# Autodesk Inventor assembly: front-tower
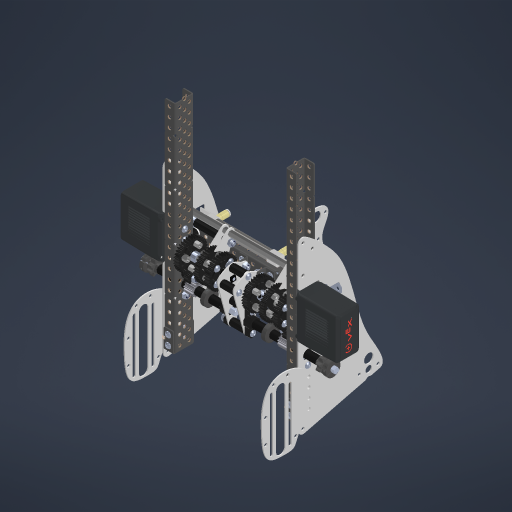
[picture p0: Inventor's stored thumbnail of the model, 512x512]
Saved by Autodesk Inventor 2023 (Build 270158000, 158)
## iProperties
Created: 2023-04-01
Part Number: front-tower
Document SubType Name: Assembly
Designer: Liam
Author: Liam
## Documents named in this file (64)
- C:\Users\eduar\VRC\CAD\Robots\Spin Up\V3\front-tower.iam
- C:\Users\eduar\VRC\CAD\Parts\standard\Structure\C-Channels\1x2x1\C-Channel 1x2x1x23.ipt
- C:\Users\eduar\VRC\CAD\Parts\standard\Structure\U-Channels\U-Channel 2x2x2x1.ipt
- C:\Users\eduar\VRC\CAD\Parts\standard\Structure\Connectors\Nut Thin Nylock.ipt
- C:\Users\eduar\VRC\CAD\Parts\standard\Structure\Connectors\Screw Steel - Star\SScrew Star Smooth .375.ipt
- C:\Users\eduar\VRC\CAD\Parts\custom\plastic\outer-tower-support-proto.ipt
- C:\Users\eduar\VRC\CAD\Parts\custom\plastic\first-stage.ipt
- C:\Users\eduar\VRC\CAD\Parts\standard\Electronics\V5 Motor.ipt
- C:\Users\eduar\VRC\CAD\Parts\standard\Structure\C-Channels\1x2x1\C-Channel 1x2x1x14.ipt
- C:\Users\eduar\VRC\CAD\Parts\standard\Motion\Spacers\Spacer Nylon .375 OD\NSpacer .375 OD x .375.ipt
- C:\Users\eduar\VRC\CAD\Parts\standard\Structure\Connectors\Screw Steel - Star\SScrew Star Smooth .750.ipt
- C:\Users\eduar\VRC\CAD\Parts\standard\Motion\Spacers\Washer Teflon\TWasher .375 OD x .06250.ipt
- C:\Users\eduar\VRC\CAD\Parts\custom\plastic\coffin-v2.ipt
- C:\Users\eduar\VRC\CAD\Parts\standard\Structure\L-Channels\L-Channel 1x1x2.ipt
- C:\Users\eduar\VRC\CAD\Parts\standard\Motion\Adapters\Insert Circle.ipt
- C:\Users\eduar\VRC\CAD\Parts\standard\Motion\Shafts\Shaft LS\Shaft LS 3.0.ipt
- C:\Users\eduar\VRC\CAD\Parts\standard\Motion\Bearings\HS Bearing Flat.ipt
- C:\Users\eduar\VRC\CAD\Parts\standard\Motion\Spacers\Spacer Nylon .375 OD\NSpacer .375 OD x .500.ipt
- C:\Users\eduar\VRC\CAD\Parts\standard\Motion\Spacers\Spacer Nylon .375 OD\NSpacer .375 OD x .250.ipt
- C:\Users\eduar\VRC\CAD\Parts\standard\Motion\Spacers\Washer Teflon\TWasher .375 OD x .04000.ipt
- C:\Users\eduar\VRC\CAD\Parts\standard\Structure\Connectors\Screw Steel - Star\SScrew Star Smooth 1.000.ipt
- C:\Users\eduar\VRC\CAD\Parts\standard\Structure\Connectors\Screw Steel - Star\SScrew Star Smooth 1.500.ipt
- C:\Users\eduar\VRC\CAD\Parts\standard\Motion\Spacers\Spacer Nylon .500 OD\NSpacer White .500 OD x .125.ipt
- C:\Users\eduar\VRC\CAD\Parts\custom\vex\Thin HS 36T Gear, No Insert.ipt
- C:\Users\eduar\VRC\CAD\Parts\standard\Motion\Adapters\Insert Square.ipt
- C:\Users\eduar\VRC\CAD\Parts\standard\Motion\Shafts\Shaft Collar\Shaft Collar Set Screw.iam
- C:\Users\eduar\VRC\CAD\Parts\standard\Motion\Gears\LS\LS 36T Gear.ipt
- C:\Users\eduar\VRC\CAD\Parts\standard\Structure\Standoff\Standoff .25.ipt
- C:\Users\eduar\VRC\CAD\Parts\standard\Motion\Spacers\Washer Teflon\TWasher .375 OD x .03125.ipt
- C:\Users\eduar\VRC\CAD\Parts\standard\Structure\Connectors\Coupler\Coupler Star .5.ipt
- C:\Users\eduar\VRC\CAD\Parts\custom\plastic\gear-interface-v3.ipt
- C:\Users\eduar\VRC\CAD\Parts\standard\Structure\Standoff\Standoff 6.00.ipt
- C:\Users\eduar\VRC\CAD\Parts\standard\Structure\Standoff\Standoff 1.00.ipt
- C:\Users\eduar\VRC\CAD\Parts\standard\Motion\Pneumatics\Reference Parts\Pistons\Double Acting Piston Body.ipt
- C:\Users\eduar\VRC\CAD\Parts\standard\Motion\Pneumatics\Reference Parts\Pistons\Double Acting Piston Rod.ipt
- C:\Users\eduar\VRC\CAD\Parts\standard\Motion\Pneumatics\Cylinder Mount.ipt
- C:\Users\eduar\VRC\CAD\Parts\standard\Motion\Pneumatics\Fitting for Cylinders.ipt
- C:\Users\eduar\VRC\CAD\Parts\standard\Motion\Shafts\Shaft Collar\Shaft Collar No Screw.iam
- C:\Users\eduar\VRC\CAD\Parts\standard\Structure\Connectors\Screw Steel - Star\SScrew Star Smooth 2.250.ipt
- C:\Users\eduar\VRC\CAD\Parts\standard\Structure\Connectors\Screw Steel - Star\SScrew Star Smooth .250.ipt
- C:\Users\eduar\VRC\CAD\Parts\standard\Motion\Spacers\Spacer Nylon .375 OD\NSpacer .375 OD x .125.ipt
- C:\Users\eduar\VRC\CAD\Parts\standard\Structure\Connectors\Screw Steel - Star\SScrew Star Smooth .875.ipt
- C:\Users\eduar\VRC\CAD\Parts\standard\Motion\Gears\LS\LS 12T Gear.ipt
- C:\Users\eduar\VRC\CAD\Parts\standard\Motion\Gears\HS\HS 12T Gear, No Insert.iam
- D:\CAD\Parts\standard\Motion\Gears\HS\HS Gear.iam
- C:\Users\eduar\VRC\CAD\Parts\standard\Motion\Spacers\HS Spacer\HSpacer .0625.ipt
- C:\Users\eduar\VRC\CAD\Parts\standard\Motion\Spacers\HS Spacer\HSpacer .1250.ipt
- C:\Users\eduar\VRC\CAD\Parts\standard\Motion\Shafts\Shaft HS\Shaft HS 5.0 in.ipt
- C:\Users\eduar\VRC\CAD\Parts\standard\Motion\Chain\6P Sprocket\6P 8T Sprocket, No Insert.iam
- C:\Users\eduar\VRC\CAD\Parts\standard\Motion\Spacers\HS Spacer\HSpacer .5000.ipt
- C:\Users\eduar\VRC\CAD\Parts\standard\Motion\Spacers\HS Spacer\HSpacer .2500.ipt
- C:\Users\eduar\VRC\CAD\Parts\standard\Motion\Shafts\Low Profile HS Shaft Collar.ipt
- C:\Users\eduar\VRC\CAD\Parts\custom\plastic\third-stage.ipt
- C:\Users\eduar\VRC\CAD\Parts\standard\Structure\Connectors\Screw Steel - Star.ipt
- C:\Users\eduar\VRC\CAD\Parts\standard\Motion\Spacers\Spacer Nylon .375 OD.ipt
- C:\Users\eduar\VRC\CAD\Parts\standard\Motion\Spacers\Washer Teflon.ipt
- C:\Users\eduar\VRC\CAD\Parts\standard\Motion\Shafts\Shaft LS.ipt
- C:\Users\eduar\VRC\CAD\Parts\standard\Motion\Spacers\Spacer Nylon .500 OD.ipt
- C:\Users\eduar\VRC\CAD\Parts\standard\Motion\Shafts\Shaft Collar.iam
- C:\Users\eduar\VRC\CAD\Parts\standard\Structure\Standoff.ipt
- C:\Users\eduar\VRC\CAD\Parts\standard\Structure\Connectors\Coupler.ipt
- C:\Users\eduar\VRC\CAD\Parts\standard\Motion\Shafts\Shaft HS.ipt
- C:\Users\eduar\VRC\CAD\Parts\standard\Motion\Spacers\HS Spacer.ipt
- C:\Users\eduar\VRC\CAD\Parts\standard\Motion\Chain\6P Sprocket.iam
## Components (262 placed, 51 different names)
1. C-Channel 1x2x1x23:1 — Rigid:1, Rigid:2, Rigid:3, Rigid:4, Rigid:5, Rigid:10, Rigid:12, Rigid:15, Rigid:17, Rigid:18, Rigid:29, Rigid:34, Rigid:35, Rigid:134, Mate:3, Mate:4, Rigid:224, Rigid:226, Rotational:14, Rigid:235
2. U-Channel 2x2x2x1:2 — Rigid:1, Rigid:6, Rigid:7, Rigid:8, Rigid:9
3. Nut Thin Nylock:1 — Rigid:3
4. Nut Thin Nylock:2 — Rigid:2
5. Nut Thin Nylock:3 — Rigid:4
6. Nut Thin Nylock:4 — Rigid:5
7. SScrew Star Smooth .375:1 — Rigid:6
8. SScrew Star Smooth .375:2 — Rigid:8
9. SScrew Star Smooth .375:3 — Rigid:7
10. SScrew Star Smooth .375:4 — Rigid:9
11. outer-tower-support-proto:1 — Rigid:10, Rigid:178, Rigid:179, Angle:3, Rigid:228, Rigid:241, Rigid:266
12. C-Channel 1x2x1x23:2 — Rigid:12, Rigid:13, Rigid:16, Rigid:19, Rigid:20, Rigid:36, Rigid:37, Rigid:42, Rigid:43, Rigid:44, Rigid:45, Rigid:46, Rigid:100, Mate:1, Mate:2, Rigid:215, Rigid:232, Rotational:13, Rigid:236
13. outer-tower-support-proto:2 — Rigid:13, Rotational:7, Rigid:180, Rigid:230, Rigid:242, Rigid:265
14. V5 Motor:1 — Rigid:16
15. V5 Motor:2 — Rigid:15
16. SScrew Star Smooth .375:5 — Rigid:17
17. SScrew Star Smooth .375:6 — Rigid:18
18. SScrew Star Smooth .375:7 — Rigid:19
19. SScrew Star Smooth .375:8 — Rigid:20
20. C-Channel 1x2x1x14:1 — Rigid:29, Rigid:30, Rigid:31, Rigid:32, Rigid:33, Rigid:47, Rigid:48, Rigid:63, Rigid:64, Rigid:65, Rigid:66, Angle:4, Rigid:263
21. Nut Thin Nylock:5
22. Nut Thin Nylock:6
23. Nut Thin Nylock:7
24. Nut Thin Nylock:8
25. NSpacer .375 OD x .375:1
26. SScrew Star Smooth .750:9 — Rigid:34
27. SScrew Star Smooth .750:10 — Rigid:35
28. SScrew Star Smooth .750:11 — Rigid:36
29. SScrew Star Smooth .750:12 — Rigid:37
30. TWasher .375 OD x .06250:1 — Rigid:30
31. NSpacer .375 OD x .375:2
32. TWasher .375 OD x .06250:2 — Rigid:33
33. NSpacer .375 OD x .375:3
34. TWasher .375 OD x .06250:3 — Rigid:32
35. NSpacer .375 OD x .375:4
36. TWasher .375 OD x .06250:4 — Rigid:31
37. U-Channel 2x2x2x1:3 — Rigid:42
38. Nut Thin Nylock:9 — Rigid:44
39. Nut Thin Nylock:10 — Rigid:43
40. Nut Thin Nylock:11 — Rigid:45
41. Nut Thin Nylock:12 — Rigid:46
42. SScrew Star Smooth .375:13
43. SScrew Star Smooth .375:14
44. SScrew Star Smooth .375:15
45. SScrew Star Smooth .375:16
46. coffin-v2:1 — Rigid:50, Rigid:61, Rigid:67, Rigid:69, Rigid:202, Rigid:203, Rigid:204, Rigid:207, Rigid:208, Rigid:209, Rigid:210, Rigid:213, Rigid:214
47. coffin-v2:2 — Rigid:49, Rigid:68, Rigid:70, Rigid:74, Rigid:75, Rigid:76, Rigid:211, Rigid:212
48. L-Channel 1x1x2:1 — Rigid:47, Rigid:50, Rigid:51, Rigid:52, Rigid:53, Rigid:54
49. L-Channel 1x1x2:2 — Rigid:48, Rigid:49, Rigid:55, Rigid:56, Rigid:57, Rigid:58
50. SScrew Star Smooth .375:17 — Rigid:52
51. SScrew Star Smooth .375:18 — Rigid:54
52. SScrew Star Smooth .375:19 — Rigid:51
53. SScrew Star Smooth .375:20 — Rigid:53
54. SScrew Star Smooth .375:21 — Rigid:57
55. SScrew Star Smooth .375:22 — Rigid:58
56. SScrew Star Smooth .375:23 — Rigid:56
57. SScrew Star Smooth .375:24 — Rigid:55
58. Nut Thin Nylock:13 — Rigid:210
59. Nut Thin Nylock:14 — Rigid:61
60. Nut Thin Nylock:15 — Rigid:211
61. Nut Thin Nylock:16 — Rigid:212
62. Nut Thin Nylock:17 — Rigid:64
63. Nut Thin Nylock:18 — Rigid:66
64. Nut Thin Nylock:19 — Rigid:63
65. Nut Thin Nylock:20 — Rigid:65
66. Insert Circle:1 — Rigid:67, Rotational:2, Rigid:151
67. Insert Circle:2 — Rigid:68, Rotational:1, Rigid:122
68. Shaft LS 3.0:1 — Rotational:1, Rigid:102, Angle:1, Rigid:127
69. Shaft LS 3.0:2 — Rotational:2, Rigid:135, Angle:2, Rigid:152
70. HS Bearing Flat:1 — Rigid:69, Rigid:97, Rigid:98, Rotational:17
71. HS Bearing Flat:2 — Rigid:70, Rigid:71, Rigid:72, Rotational:18
72. Nut Thin Nylock:21 — Rigid:71
73. Nut Thin Nylock:22 — Rigid:72
74. Nut Thin Nylock:23 — Rigid:76
75. Nut Thin Nylock:24 — Rigid:75
76. Nut Thin Nylock:26 — Rigid:74
77. NSpacer .375 OD x .500:5
78. NSpacer .375 OD x .250:6
79. TWasher .375 OD x .04000:5 — Rigid:208
80. NSpacer .375 OD x .500:7
81. NSpacer .375 OD x .250:8
82. TWasher .375 OD x .04000:6 — Rigid:213
83. NSpacer .375 OD x .500:9
84. NSpacer .375 OD x .250:10
85. TWasher .375 OD x .04000:7 — Rigid:214
86. NSpacer .375 OD x .500:11
87. NSpacer .375 OD x .250:12
88. TWasher .375 OD x .04000:8 — Rigid:207
89. NSpacer .375 OD x .500:13
90. NSpacer .375 OD x .250:14
91. TWasher .375 OD x .04000:9 — Rigid:209
92. SScrew Star Smooth 1.000:25 — Rigid:202
93. SScrew Star Smooth 1.000:26 — Rigid:203
94. SScrew Star Smooth 1.000:27 — Rigid:204
95. SScrew Star Smooth 1.500:29 — Rigid:97
96. SScrew Star Smooth 1.500:30 — Rigid:98
97. NSpacer White .500 OD x .125:1 — Rigid:100
98. TWasher .375 OD x .06250:10 — Rotational:3
99. Thin HS 36T Gear, No Insert:1 — Rigid:101, Rotational:3, Rigid:103, Rigid:104, Rigid:105, Rigid:106, Rigid:153, Rigid:154, Rigid:155, Rigid:156
100. Insert Square:1 — Rigid:101
101. Shaft Collar Set Screw:1 [sub-assembly] — Rigid:102
102. LS 36T Gear:2 — Angle:1, Mate:1, Rigid:107, Rigid:108, Rigid:109, Rigid:110, Rigid:111, Rigid:112, Rigid:113, Rigid:114, Mate:2, Insert:1, Mate:6, Mate:8, Mate:9
103. Standoff .25:1 — Rigid:105
104. Standoff .25:2 — Rigid:106
105. Standoff .25:3 — Rigid:104
106. Standoff .25:4 — Rigid:112, Rigid:169
107. Standoff .25:5 — Rigid:103
108. Standoff .25:6 — Rigid:107
109. Standoff .25:7 — Rigid:111, Rigid:170
110. Standoff .25:8 — Rigid:113, Rigid:172
111. Standoff .25:9 — Rigid:109
112. Standoff .25:10 — Rigid:110
113. Standoff .25:11 — Rigid:114, Rigid:171
114. Standoff .25:12 — Rigid:108
115. Thin HS 36T Gear, No Insert:2 — Rigid:123, Rigid:124, Rigid:125, Rigid:126, Rigid:157, Rigid:158, Rigid:159, Rigid:160
116. Insert Square:2 — Rotational:4
117. NSpacer .375 OD x .250:15 — Rotational:4
118. TWasher .375 OD x .04000:11
119. TWasher .375 OD x .03125:12 — Rigid:122
120. Standoff .25:13 — Rigid:123
121. Standoff .25:14 — Rigid:126
122. Standoff .25:15 — Rigid:124
123. Standoff .25:16 — Rigid:125
124. Shaft Collar Set Screw:2 [sub-assembly] — Rigid:127
125. NSpacer White .500 OD x .125:2 — Rigid:134
126. TWasher .375 OD x .06250:13
127. Thin HS 36T Gear, No Insert:3 — Rigid:165, Rigid:166, Rigid:167, Rigid:168
128. Insert Square:3
129. Standoff .25:17
130. Standoff .25:18
131. Standoff .25:19
132. Standoff .25:20
133. Shaft Collar Set Screw:3 [sub-assembly] — Rigid:135
134. LS 36T Gear:3 — Mate:3, Angle:2, Mate:4, Mate:10, Mate:12, Mate:13, Mate:15
135. Standoff .25:21 — Rigid:174
136. Standoff .25:22
137. Standoff .25:23
138. Standoff .25:24 — Rigid:173
139. Standoff .25:25
140. Standoff .25:26
141. Standoff .25:27 — Rigid:176
142. Standoff .25:28
143. Thin HS 36T Gear, No Insert:4 — Rigid:161, Rigid:162, Rigid:163, Rigid:164
144. Insert Square:4
145. NSpacer .375 OD x .250:16
146. TWasher .375 OD x .04000:14
147. TWasher .375 OD x .03125:15 — Rigid:151
148. Standoff .25:29
149. Standoff .25:30
150. Standoff .25:31 — Rigid:175
151. Standoff .25:32
152. Shaft Collar Set Screw:4 [sub-assembly] — Rigid:152
153. SScrew Star Smooth .375:31 — Rigid:153
154. SScrew Star Smooth .375:32 — Rigid:154
155. SScrew Star Smooth .375:33 — Rigid:155
156. SScrew Star Smooth .375:34 — Rigid:156
157. SScrew Star Smooth .375:35 — Rigid:159
158. SScrew Star Smooth .375:36 — Rigid:160
159. SScrew Star Smooth .375:37 — Rigid:157
160. SScrew Star Smooth .375:38 — Rigid:158
161. SScrew Star Smooth .375:39 — Rigid:161
162. SScrew Star Smooth .375:40 — Rigid:162
163. SScrew Star Smooth .375:41 — Rigid:164
164. SScrew Star Smooth .375:42 — Rigid:163
165. SScrew Star Smooth .375:43 — Rigid:167
166. SScrew Star Smooth .375:44 — Rigid:166
167. SScrew Star Smooth .375:45 — Rigid:165
168. SScrew Star Smooth .375:46 — Rigid:168
169. Coupler Star .5:1 — Rigid:172
170. Coupler Star .5:2 — Rigid:171
171. Coupler Star .5:3 — Rigid:170
172. Coupler Star .5:4 — Rigid:169
173. Coupler Star .5:5 — Rigid:173
174. Coupler Star .5:6 — Rigid:174
175. Coupler Star .5:7 — Rigid:175
176. Coupler Star .5:8 — Rigid:176
177. gear-interface-v3:1 — Insert:1, Mate:5, Mate:9, Rigid:182, Rigid:183
178. Standoff 6.00:33 — Rotational:7, Mate:5, Mate:7, Mate:11, Mate:14, Rigid:177
179. gear-interface-v3:2 — Mate:6, Mate:7, Mate:8, Mate:20, Mate:22
180. gear-interface-v3:3 — Mate:10, Mate:11, Mate:12, Rigid:184
181. gear-interface-v3:4 — Mate:13, Mate:14, Mate:15, Rigid:181, Mate:21
182. Standoff 1.00:34 — Rigid:177
183. NSpacer White .500 OD x .125:3 — Rigid:178
184. SScrew Star Smooth .375:47 — Rigid:179
185. SScrew Star Smooth .375:48 — Rigid:180
186. NSpacer .375 OD x .250:17 — Rigid:181
187. NSpacer .375 OD x .250:18 — Rigid:182
188. Nut Thin Nylock:28 — Rigid:184
189. Nut Thin Nylock:29 — Rigid:183
190. Double Acting Piston Body:1 — Rigid:185, Rigid:186, Angle:4, Rigid:187, Rigid:199
191. Double Acting Piston Rod:1 — Rotational:8
192. Cylinder Mount:1 — Rotational:8, Angle:3, Mate:18
193. Fitting for Cylinders:1 — Rigid:185
194. Fitting for Cylinders:2 — Rigid:186
195. Shaft Collar No Screw:5 [sub-assembly] — Rigid:187, Mate:19, Mate:20, Mate:22, Rigid:189, Rigid:197
196. Shaft Collar No Screw:6 [sub-assembly] — Mate:18, Mate:19, Mate:21, Rigid:188, Rigid:192, Rigid:198
197. SScrew Star Smooth 2.250:49 — Rigid:188
198. SScrew Star Smooth 2.250:50 — Rigid:189
199. NSpacer .375 OD x .375:19 — Rigid:191, Rigid:193
200. NSpacer .375 OD x .500:20 — Rigid:190, Rigid:192
201. NSpacer .375 OD x .500:21 — Rigid:190, Rigid:191
202. TWasher .375 OD x .04000:16 — Rigid:193
203. NSpacer .375 OD x .375:22
204. NSpacer .375 OD x .500:23 — Rigid:197
205. NSpacer .375 OD x .500:24
206. TWasher .375 OD x .04000:17
207. SScrew Star Smooth .250:51 — Rigid:198
208. SScrew Star Smooth .250:52 — Rigid:199
209. HS Bearing Flat:5 — Rigid:215, Rigid:216, Rigid:219, Rigid:246
210. Nut Thin Nylock:30 — Rigid:216, Rigid:217
211. NSpacer .375 OD x .125:25 — Rigid:217
212. Nut Thin Nylock:31 — Rigid:219
213. NSpacer .375 OD x .125:26
214. HS Bearing Flat:6 — Rigid:224, Rigid:251
215. Nut Thin Nylock:32
216. NSpacer .375 OD x .125:27
217. Nut Thin Nylock:33
218. NSpacer .375 OD x .125:28
219. Nut Thin Nylock:35 — Rigid:226
220. SScrew Star Smooth .875:54 — Rigid:228
221. SScrew Star Smooth .875:56 — Rigid:230
222. Nut Thin Nylock:37 — Rigid:232
223. LS 12T Gear:1 — Rotational:13, Rotational:15
224. LS 12T Gear:2 — Rotational:14, Rotational:16
225. Nut Thin Nylock:38 — Rotational:15
226. Nut Thin Nylock:39 — Rotational:16
227. HS 12T Gear, No Insert:1 [sub-assembly] — Rigid:238, Rigid:244, Rigid:254
228. HS 12T Gear, No Insert:2 [sub-assembly] — Rigid:240, Rigid:243, Rigid:253
229. NSpacer .375 OD x .125:29 — Rigid:235
230. NSpacer .375 OD x .125:30 — Rigid:236
231. HSpacer .0625:1 — Rigid:237
232. HSpacer .1250:2 — Rigid:237, Rigid:238
233. HSpacer .0625:3
234. HSpacer .1250:4 — Rigid:240
235. SScrew Star Smooth 1.500:57 — Rigid:242
236. SScrew Star Smooth 1.500:58 — Rigid:241
237. Shaft HS 5.0 in:2 — Rotational:17, Rigid:244, Rigid:250, Rigid:252
238. Shaft HS 5.0 in:3 — Rotational:18, Rigid:243, Rigid:245, Rigid:248
239. 6P 8T Sprocket, No Insert:1 [sub-assembly] — Rigid:245
240. HSpacer .5000:5 — Rigid:246, Rigid:247
241. HSpacer .2500:6 — Rigid:247, Rotational:19
242. HSpacer .1250:7 — Rotational:19
243. Low Profile HS Shaft Collar:1 — Rigid:248
244. 6P 8T Sprocket, No Insert:2 [sub-assembly] — Rigid:250
245. HSpacer .5000:8 — Rigid:251
246. HSpacer .2500:9
247. HSpacer .1250:10
248. Low Profile HS Shaft Collar:2 — Rigid:252
249. HSpacer .5000:11 — Rigid:253, Rigid:255
250. HSpacer .5000:12 — Rigid:254, Rigid:256
251. Low Profile HS Shaft Collar:3 — Rigid:255, Rigid:257
252. Low Profile HS Shaft Collar:4 — Rigid:256, Rigid:262
253. HSpacer .5000:13 — Rigid:257, Rigid:258
254. HSpacer .1250:14 — Rigid:258, Rigid:259
255. HSpacer .0625:15 — Rigid:259
256. HSpacer .5000:16 — Rigid:262
257. HSpacer .1250:17
258. HSpacer .0625:18
259. L-Channel 1x1x2:3 — Rigid:263, Rigid:264
260. third-stage:1 — Rigid:264
261. first-stage:3 — Rigid:265
262. first-stage:4 — Rigid:266
## Relationships (279: WeldJoint 236, Mate 22, RevoluteJoint 16, Angle 4, Insert 1)
- Rigid:1 [WeldJoint]: C-Channel 1x2x1x23:1 ↔ U-Channel 2x2x2x1:2
- Rigid:2 [WeldJoint]: C-Channel 1x2x1x23:1 ↔ Nut Thin Nylock:2
- Rigid:3 [WeldJoint]: C-Channel 1x2x1x23:1 ↔ Nut Thin Nylock:1
- Rigid:4 [WeldJoint]: C-Channel 1x2x1x23:1 ↔ Nut Thin Nylock:3
- Rigid:5 [WeldJoint]: C-Channel 1x2x1x23:1 ↔ Nut Thin Nylock:4
- Rigid:6 [WeldJoint]: U-Channel 2x2x2x1:2 ↔ SScrew Star Smooth .375:1
- Rigid:7 [WeldJoint]: U-Channel 2x2x2x1:2 ↔ SScrew Star Smooth .375:3
- Rigid:8 [WeldJoint]: U-Channel 2x2x2x1:2 ↔ SScrew Star Smooth .375:2
- Rigid:9 [WeldJoint]: U-Channel 2x2x2x1:2 ↔ SScrew Star Smooth .375:4
- Rigid:10 [WeldJoint] (14.2875 mm): C-Channel 1x2x1x23:1 ↔ outer-tower-support-proto:1
- Rigid:12 [WeldJoint] (149.225 mm): C-Channel 1x2x1x23:1 ↔ C-Channel 1x2x1x23:2
- Rigid:13 [WeldJoint] (14.2875 mm): C-Channel 1x2x1x23:2 ↔ outer-tower-support-proto:2
- Rigid:15 [WeldJoint]: C-Channel 1x2x1x23:1 ↔ V5 Motor:2
- Rigid:16 [WeldJoint]: C-Channel 1x2x1x23:2 ↔ V5 Motor:1
- Rigid:17 [WeldJoint]: C-Channel 1x2x1x23:1 ↔ SScrew Star Smooth .375:5
- Rigid:18 [WeldJoint]: C-Channel 1x2x1x23:1 ↔ SScrew Star Smooth .375:6
- Rigid:19 [WeldJoint]: C-Channel 1x2x1x23:2 ↔ SScrew Star Smooth .375:7
- Rigid:20 [WeldJoint]: C-Channel 1x2x1x23:2 ↔ SScrew Star Smooth .375:8
- [WeldJoint]: C-Channel 1x2x1x14:1 ↔ Nut Thin Nylock:5
- [WeldJoint]: C-Channel 1x2x1x14:1 ↔ Nut Thin Nylock:6
- [WeldJoint]: C-Channel 1x2x1x14:1 ↔ Nut Thin Nylock:7
- [WeldJoint]: C-Channel 1x2x1x14:1 ↔ Nut Thin Nylock:8
- [WeldJoint]: NSpacer .375 OD x .375:1 ↔ TWasher .375 OD x .06250:1
- [WeldJoint]: NSpacer .375 OD x .375:2 ↔ TWasher .375 OD x .06250:2
- [WeldJoint]: NSpacer .375 OD x .375:3 ↔ TWasher .375 OD x .06250:3
- [WeldJoint]: NSpacer .375 OD x .375:4 ↔ TWasher .375 OD x .06250:4
- Rigid:29 [WeldJoint] (11.1125 mm): C-Channel 1x2x1x23:1 ↔ C-Channel 1x2x1x14:1
- Rigid:30 [WeldJoint]: C-Channel 1x2x1x14:1 ↔ TWasher .375 OD x .06250:1
- Rigid:31 [WeldJoint]: C-Channel 1x2x1x14:1 ↔ TWasher .375 OD x .06250:4
- Rigid:32 [WeldJoint]: C-Channel 1x2x1x14:1 ↔ TWasher .375 OD x .06250:3
- Rigid:33 [WeldJoint]: C-Channel 1x2x1x14:1 ↔ TWasher .375 OD x .06250:2
- Rigid:34 [WeldJoint]: C-Channel 1x2x1x23:1 ↔ SScrew Star Smooth .750:9
- Rigid:35 [WeldJoint]: C-Channel 1x2x1x23:1 ↔ SScrew Star Smooth .750:10
- Rigid:36 [WeldJoint]: C-Channel 1x2x1x23:2 ↔ SScrew Star Smooth .750:11
- Rigid:37 [WeldJoint]: C-Channel 1x2x1x23:2 ↔ SScrew Star Smooth .750:12
- [WeldJoint]: U-Channel 2x2x2x1:3 ↔ SScrew Star Smooth .375:13
- [WeldJoint]: U-Channel 2x2x2x1:3 ↔ SScrew Star Smooth .375:15
- [WeldJoint]: U-Channel 2x2x2x1:3 ↔ SScrew Star Smooth .375:14
- [WeldJoint]: U-Channel 2x2x2x1:3 ↔ SScrew Star Smooth .375:16
- Rigid:42 [WeldJoint]: C-Channel 1x2x1x23:2 ↔ U-Channel 2x2x2x1:3
- Rigid:43 [WeldJoint]: C-Channel 1x2x1x23:2 ↔ Nut Thin Nylock:10
- Rigid:44 [WeldJoint]: C-Channel 1x2x1x23:2 ↔ Nut Thin Nylock:9
- Rigid:45 [WeldJoint]: C-Channel 1x2x1x23:2 ↔ Nut Thin Nylock:11
- Rigid:46 [WeldJoint]: C-Channel 1x2x1x23:2 ↔ Nut Thin Nylock:12
- Rigid:47 [WeldJoint]: C-Channel 1x2x1x14:1 ↔ L-Channel 1x1x2:1
- Rigid:48 [WeldJoint]: C-Channel 1x2x1x14:1 ↔ L-Channel 1x1x2:2
- Rigid:49 [WeldJoint]: coffin-v2:2 ↔ L-Channel 1x1x2:2
- Rigid:50 [WeldJoint]: coffin-v2:1 ↔ L-Channel 1x1x2:1
- Rigid:51 [WeldJoint]: L-Channel 1x1x2:1 ↔ SScrew Star Smooth .375:19
- Rigid:52 [WeldJoint]: L-Channel 1x1x2:1 ↔ SScrew Star Smooth .375:17
- Rigid:53 [WeldJoint]: L-Channel 1x1x2:1 ↔ SScrew Star Smooth .375:20
- Rigid:54 [WeldJoint]: L-Channel 1x1x2:1 ↔ SScrew Star Smooth .375:18
- Rigid:55 [WeldJoint]: L-Channel 1x1x2:2 ↔ SScrew Star Smooth .375:24
- Rigid:56 [WeldJoint]: L-Channel 1x1x2:2 ↔ SScrew Star Smooth .375:23
- Rigid:57 [WeldJoint]: L-Channel 1x1x2:2 ↔ SScrew Star Smooth .375:21
- Rigid:58 [WeldJoint]: L-Channel 1x1x2:2 ↔ SScrew Star Smooth .375:22
- Rigid:61 [WeldJoint]: coffin-v2:1 ↔ Nut Thin Nylock:14
- Rigid:63 [WeldJoint]: C-Channel 1x2x1x14:1 ↔ Nut Thin Nylock:19
- Rigid:64 [WeldJoint]: C-Channel 1x2x1x14:1 ↔ Nut Thin Nylock:17
- Rigid:65 [WeldJoint]: C-Channel 1x2x1x14:1 ↔ Nut Thin Nylock:20
- Rigid:66 [WeldJoint]: C-Channel 1x2x1x14:1 ↔ Nut Thin Nylock:18
- Rigid:67 [WeldJoint]: coffin-v2:1 ↔ Insert Circle:1
- Rigid:68 [WeldJoint]: coffin-v2:2 ↔ Insert Circle:2
- Rotational:1 [RevoluteJoint]: Insert Circle:2 ↔ Shaft LS 3.0:1
- Rotational:2 [RevoluteJoint]: Insert Circle:1 ↔ Shaft LS 3.0:2
- Rigid:69 [WeldJoint]: coffin-v2:1 ↔ HS Bearing Flat:1
- Rigid:70 [WeldJoint]: coffin-v2:2 ↔ HS Bearing Flat:2
- Rigid:71 [WeldJoint]: HS Bearing Flat:2 ↔ Nut Thin Nylock:21
- Rigid:72 [WeldJoint]: HS Bearing Flat:2 ↔ Nut Thin Nylock:22
- Rigid:74 [WeldJoint]: coffin-v2:2 ↔ Nut Thin Nylock:26
- Rigid:75 [WeldJoint]: coffin-v2:2 ↔ Nut Thin Nylock:24
- Rigid:76 [WeldJoint]: coffin-v2:2 ↔ Nut Thin Nylock:23
- [WeldJoint]: NSpacer .375 OD x .500:5 ↔ NSpacer .375 OD x .250:6
- [WeldJoint]: NSpacer .375 OD x .250:6 ↔ TWasher .375 OD x .04000:5
- [WeldJoint]: NSpacer .375 OD x .500:7 ↔ NSpacer .375 OD x .250:8
- [WeldJoint]: NSpacer .375 OD x .250:8 ↔ TWasher .375 OD x .04000:6
- [WeldJoint]: NSpacer .375 OD x .500:9 ↔ NSpacer .375 OD x .250:10
- [WeldJoint]: NSpacer .375 OD x .250:10 ↔ TWasher .375 OD x .04000:7
- [WeldJoint]: NSpacer .375 OD x .500:11 ↔ NSpacer .375 OD x .250:12
- [WeldJoint]: NSpacer .375 OD x .250:12 ↔ TWasher .375 OD x .04000:8
- [WeldJoint]: NSpacer .375 OD x .500:13 ↔ NSpacer .375 OD x .250:14
- [WeldJoint]: NSpacer .375 OD x .250:14 ↔ TWasher .375 OD x .04000:9
- Rigid:97 [WeldJoint]: HS Bearing Flat:1 ↔ SScrew Star Smooth 1.500:29
- Rigid:98 [WeldJoint]: HS Bearing Flat:1 ↔ SScrew Star Smooth 1.500:30
- [WeldJoint]: NSpacer White .500 OD x .125:1 ↔ TWasher .375 OD x .06250:10
- Rigid:100 [WeldJoint]: C-Channel 1x2x1x23:2 ↔ NSpacer White .500 OD x .125:1
- Rigid:101 [WeldJoint] (-3.175 mm): Thin HS 36T Gear, No Insert:1 ↔ Insert Square:1
- Rotational:3 [RevoluteJoint] (3.175 mm): TWasher .375 OD x .06250:10 ↔ Thin HS 36T Gear, No Insert:1
- Rigid:102 [WeldJoint] (-54.5084 mm): Shaft LS 3.0:1 ↔ Shaft Collar Set Screw:1
- Angle:1 (0 deg): Shaft LS 3.0:1 ↔ LS 36T Gear:2
- Mate:1: C-Channel 1x2x1x23:2 ↔ LS 36T Gear:2
- Rigid:103 [WeldJoint]: Thin HS 36T Gear, No Insert:1 ↔ Standoff .25:5
- Rigid:104 [WeldJoint]: Thin HS 36T Gear, No Insert:1 ↔ Standoff .25:3
- Rigid:105 [WeldJoint]: Thin HS 36T Gear, No Insert:1 ↔ Standoff .25:1
- Rigid:106 [WeldJoint]: Thin HS 36T Gear, No Insert:1 ↔ Standoff .25:2
- Rigid:107 [WeldJoint]: LS 36T Gear:2 ↔ Standoff .25:6
- Rigid:108 [WeldJoint]: LS 36T Gear:2 ↔ Standoff .25:12
- Rigid:109 [WeldJoint]: LS 36T Gear:2 ↔ Standoff .25:9
- Rigid:110 [WeldJoint]: LS 36T Gear:2 ↔ Standoff .25:10
- Rigid:111 [WeldJoint]: LS 36T Gear:2 ↔ Standoff .25:7
- Rigid:112 [WeldJoint]: LS 36T Gear:2 ↔ Standoff .25:4
- Rigid:113 [WeldJoint]: LS 36T Gear:2 ↔ Standoff .25:8
- Rigid:114 [WeldJoint]: LS 36T Gear:2 ↔ Standoff .25:11
- [WeldJoint] (-3.175 mm): Thin HS 36T Gear, No Insert:2 ↔ Insert Square:2
- [WeldJoint]: TWasher .375 OD x .04000:11 ↔ TWasher .375 OD x .03125:12
- [WeldJoint]: NSpacer .375 OD x .250:15 ↔ TWasher .375 OD x .04000:11
- Rigid:122 [WeldJoint]: Insert Circle:2 ↔ TWasher .375 OD x .03125:12
- Rotational:4 [RevoluteJoint]: Insert Square:2 ↔ NSpacer .375 OD x .250:15
- Rigid:123 [WeldJoint]: Thin HS 36T Gear, No Insert:2 ↔ Standoff .25:13
- Rigid:124 [WeldJoint]: Thin HS 36T Gear, No Insert:2 ↔ Standoff .25:15
- Rigid:125 [WeldJoint]: Thin HS 36T Gear, No Insert:2 ↔ Standoff .25:16
- Rigid:126 [WeldJoint]: Thin HS 36T Gear, No Insert:2 ↔ Standoff .25:14
- Rigid:127 [WeldJoint] (-20.8534 mm): Shaft LS 3.0:1 ↔ Shaft Collar Set Screw:2
- Mate:2: C-Channel 1x2x1x23:2 ↔ LS 36T Gear:2
- [WeldJoint]: NSpacer White .500 OD x .125:2 ↔ TWasher .375 OD x .06250:13
- [WeldJoint] (-3.175 mm): Thin HS 36T Gear, No Insert:3 ↔ Insert Square:3
- [RevoluteJoint] (3.175 mm): TWasher .375 OD x .06250:13 ↔ Thin HS 36T Gear, No Insert:3
- [WeldJoint]: Thin HS 36T Gear, No Insert:3 ↔ Standoff .25:20
- [WeldJoint]: Thin HS 36T Gear, No Insert:3 ↔ Standoff .25:19
- [WeldJoint]: Thin HS 36T Gear, No Insert:3 ↔ Standoff .25:17
- [WeldJoint]: Thin HS 36T Gear, No Insert:3 ↔ Standoff .25:18
- Rigid:134 [WeldJoint]: C-Channel 1x2x1x23:1 ↔ NSpacer White .500 OD x .125:2
- Rigid:135 [WeldJoint] (-54.5084 mm): Shaft LS 3.0:2 ↔ Shaft Collar Set Screw:3
- [WeldJoint]: LS 36T Gear:3 ↔ Standoff .25:22
- [WeldJoint]: LS 36T Gear:3 ↔ Standoff .25:28
- [WeldJoint]: LS 36T Gear:3 ↔ Standoff .25:25
- [WeldJoint]: LS 36T Gear:3 ↔ Standoff .25:26
- [WeldJoint]: LS 36T Gear:3 ↔ Standoff .25:23
- [WeldJoint]: LS 36T Gear:3 ↔ Standoff .25:21
- [WeldJoint]: LS 36T Gear:3 ↔ Standoff .25:24
- [WeldJoint]: LS 36T Gear:3 ↔ Standoff .25:27
- Mate:3: C-Channel 1x2x1x23:1 ↔ LS 36T Gear:3
- Angle:2 (0 deg): Shaft LS 3.0:2 ↔ LS 36T Gear:3
- Mate:4: C-Channel 1x2x1x23:1 ↔ LS 36T Gear:3
- [WeldJoint] (-3.175 mm): Thin HS 36T Gear, No Insert:4 ↔ Insert Square:4
- [WeldJoint]: TWasher .375 OD x .04000:14 ↔ TWasher .375 OD x .03125:15
- [WeldJoint]: NSpacer .375 OD x .250:16 ↔ TWasher .375 OD x .04000:14
- [RevoluteJoint]: Insert Square:4 ↔ NSpacer .375 OD x .250:16
- [WeldJoint]: Thin HS 36T Gear, No Insert:4 ↔ Standoff .25:29
- [WeldJoint]: Thin HS 36T Gear, No Insert:4 ↔ Standoff .25:31
- [WeldJoint]: Thin HS 36T Gear, No Insert:4 ↔ Standoff .25:32
- [WeldJoint]: Thin HS 36T Gear, No Insert:4 ↔ Standoff .25:30
- Rigid:151 [WeldJoint]: Insert Circle:1 ↔ TWasher .375 OD x .03125:15
- Rigid:152 [WeldJoint] (-27.2034 mm): Shaft LS 3.0:2 ↔ Shaft Collar Set Screw:4
- Rigid:153 [WeldJoint]: Thin HS 36T Gear, No Insert:1 ↔ SScrew Star Smooth .375:31
- Rigid:154 [WeldJoint]: Thin HS 36T Gear, No Insert:1 ↔ SScrew Star Smooth .375:32
- Rigid:155 [WeldJoint]: Thin HS 36T Gear, No Insert:1 ↔ SScrew Star Smooth .375:33
- Rigid:156 [WeldJoint]: Thin HS 36T Gear, No Insert:1 ↔ SScrew Star Smooth .375:34
- Rigid:157 [WeldJoint]: Thin HS 36T Gear, No Insert:2 ↔ SScrew Star Smooth .375:37
- Rigid:158 [WeldJoint]: Thin HS 36T Gear, No Insert:2 ↔ SScrew Star Smooth .375:38
- Rigid:159 [WeldJoint]: Thin HS 36T Gear, No Insert:2 ↔ SScrew Star Smooth .375:35
- Rigid:160 [WeldJoint]: Thin HS 36T Gear, No Insert:2 ↔ SScrew Star Smooth .375:36
- Rigid:161 [WeldJoint]: Thin HS 36T Gear, No Insert:4 ↔ SScrew Star Smooth .375:39
- Rigid:162 [WeldJoint]: Thin HS 36T Gear, No Insert:4 ↔ SScrew Star Smooth .375:40
- Rigid:163 [WeldJoint]: Thin HS 36T Gear, No Insert:4 ↔ SScrew Star Smooth .375:42
- Rigid:164 [WeldJoint]: Thin HS 36T Gear, No Insert:4 ↔ SScrew Star Smooth .375:41
- Rigid:165 [WeldJoint]: Thin HS 36T Gear, No Insert:3 ↔ SScrew Star Smooth .375:45
- Rigid:166 [WeldJoint]: Thin HS 36T Gear, No Insert:3 ↔ SScrew Star Smooth .375:44
- Rigid:167 [WeldJoint]: Thin HS 36T Gear, No Insert:3 ↔ SScrew Star Smooth .375:43
- Rigid:168 [WeldJoint]: Thin HS 36T Gear, No Insert:3 ↔ SScrew Star Smooth .375:46
- Rigid:169 [WeldJoint] (-1 mm): Standoff .25:4 ↔ Coupler Star .5:4
- Rigid:170 [WeldJoint] (-1 mm): Standoff .25:7 ↔ Coupler Star .5:3
- Rigid:171 [WeldJoint] (-1 mm): Standoff .25:11 ↔ Coupler Star .5:2
- Rigid:172 [WeldJoint] (-1 mm): Standoff .25:8 ↔ Coupler Star .5:1
- Rigid:173 [WeldJoint] (-1 mm): Standoff .25:24 ↔ Coupler Star .5:5
- Rigid:174 [WeldJoint] (-1 mm): Standoff .25:21 ↔ Coupler Star .5:6
- Rigid:175 [WeldJoint] (1 mm): Standoff .25:31 ↔ Coupler Star .5:7
- Rigid:176 [WeldJoint] (-1 mm): Standoff .25:27 ↔ Coupler Star .5:8
- Insert:1: LS 36T Gear:2 ↔ gear-interface-v3:1
- Rotational:7 [RevoluteJoint]: outer-tower-support-proto:2 ↔ Standoff 6.00:33
- Mate:5: gear-interface-v3:1 ↔ Standoff 6.00:33
- Mate:6: LS 36T Gear:2 ↔ gear-interface-v3:2
- Mate:7: Standoff 6.00:33 ↔ gear-interface-v3:2
- Mate:8: LS 36T Gear:2 ↔ gear-interface-v3:2
- Mate:9: LS 36T Gear:2 ↔ gear-interface-v3:1
- Mate:10: LS 36T Gear:3 ↔ gear-interface-v3:3
- Mate:11: Standoff 6.00:33 ↔ gear-interface-v3:3
- Mate:12: LS 36T Gear:3 ↔ gear-interface-v3:3
- Mate:13: LS 36T Gear:3 ↔ gear-interface-v3:4
- Mate:14: Standoff 6.00:33 ↔ gear-interface-v3:4
- Mate:15: LS 36T Gear:3 ↔ gear-interface-v3:4
- Rigid:177 [WeldJoint]: Standoff 6.00:33 ↔ Standoff 1.00:34
- Rigid:178 [WeldJoint]: outer-tower-support-proto:1 ↔ NSpacer White .500 OD x .125:3
- Rigid:179 [WeldJoint]: outer-tower-support-proto:1 ↔ SScrew Star Smooth .375:47
- Rigid:180 [WeldJoint]: outer-tower-support-proto:2 ↔ SScrew Star Smooth .375:48
- Rigid:181 [WeldJoint]: gear-interface-v3:4 ↔ NSpacer .375 OD x .250:17
- Rigid:182 [WeldJoint]: gear-interface-v3:1 ↔ NSpacer .375 OD x .250:18
- Rigid:183 [WeldJoint]: gear-interface-v3:1 ↔ Nut Thin Nylock:29
- Rigid:184 [WeldJoint]: gear-interface-v3:3 ↔ Nut Thin Nylock:28
- [Mate]: Double Acting Piston Body:1 ↔ Double Acting Piston Rod:1
- [Mate]: Double Acting Piston Body:1 ↔ Double Acting Piston Rod:1
- Rotational:8 [RevoluteJoint] (7.62 mm): Double Acting Piston Rod:1 ↔ Cylinder Mount:1
- Rigid:185 [WeldJoint]: Double Acting Piston Body:1 ↔ Fitting for Cylinders:1
- Rigid:186 [WeldJoint]: Double Acting Piston Body:1 ↔ Fitting for Cylinders:2
- Angle:3 (0 deg): outer-tower-support-proto:1 ↔ Cylinder Mount:1
- Angle:4 (0 deg): C-Channel 1x2x1x14:1 ↔ Double Acting Piston Body:1
- Rigid:187 [WeldJoint]: Double Acting Piston Body:1 ↔ Shaft Collar No Screw:5
- Mate:18: Cylinder Mount:1 ↔ Shaft Collar No Screw:6
- Mate:19: Shaft Collar No Screw:5 ↔ Shaft Collar No Screw:6
- Mate:20: gear-interface-v3:2 ↔ Shaft Collar No Screw:5
- Mate:21 (36.1122 mm): gear-interface-v3:4 ↔ Shaft Collar No Screw:6
- Mate:22 (36.1122 mm): gear-interface-v3:2 ↔ Shaft Collar No Screw:5
- Rigid:188 [WeldJoint]: Shaft Collar No Screw:6 ↔ SScrew Star Smooth 2.250:49
- Rigid:189 [WeldJoint]: Shaft Collar No Screw:5 ↔ SScrew Star Smooth 2.250:50
- Rigid:190 [WeldJoint]: NSpacer .375 OD x .500:20 ↔ NSpacer .375 OD x .500:21
- Rigid:191 [WeldJoint]: NSpacer .375 OD x .375:19 ↔ NSpacer .375 OD x .500:21
- Rigid:192 [WeldJoint]: Shaft Collar No Screw:6 ↔ NSpacer .375 OD x .500:20
- Rigid:193 [WeldJoint]: NSpacer .375 OD x .375:19 ↔ TWasher .375 OD x .04000:16
- [WeldJoint]: NSpacer .375 OD x .500:23 ↔ NSpacer .375 OD x .500:24
- [WeldJoint]: NSpacer .375 OD x .375:22 ↔ NSpacer .375 OD x .500:24
- [WeldJoint]: NSpacer .375 OD x .375:22 ↔ TWasher .375 OD x .04000:17
- Rigid:197 [WeldJoint]: Shaft Collar No Screw:5 ↔ NSpacer .375 OD x .500:23
- Rigid:198 [WeldJoint]: Shaft Collar No Screw:6 ↔ SScrew Star Smooth .250:51
- Rigid:199 [WeldJoint]: Double Acting Piston Body:1 ↔ SScrew Star Smooth .250:52
- Rigid:202 [WeldJoint]: coffin-v2:1 ↔ SScrew Star Smooth 1.000:25
- Rigid:203 [WeldJoint]: coffin-v2:1 ↔ SScrew Star Smooth 1.000:26
- Rigid:204 [WeldJoint]: coffin-v2:1 ↔ SScrew Star Smooth 1.000:27
- Rigid:207 [WeldJoint]: coffin-v2:1 ↔ TWasher .375 OD x .04000:8
- Rigid:208 [WeldJoint]: coffin-v2:1 ↔ TWasher .375 OD x .04000:5
- Rigid:209 [WeldJoint]: coffin-v2:1 ↔ TWasher .375 OD x .04000:9
- Rigid:210 [WeldJoint]: coffin-v2:1 ↔ Nut Thin Nylock:13
- Rigid:211 [WeldJoint]: coffin-v2:2 ↔ Nut Thin Nylock:15
- Rigid:212 [WeldJoint]: coffin-v2:2 ↔ Nut Thin Nylock:16
- Rigid:213 [WeldJoint]: coffin-v2:1 ↔ TWasher .375 OD x .04000:6
- Rigid:214 [WeldJoint]: coffin-v2:1 ↔ TWasher .375 OD x .04000:7
- Rigid:215 [WeldJoint]: C-Channel 1x2x1x23:2 ↔ HS Bearing Flat:5
- Rigid:216 [WeldJoint]: HS Bearing Flat:5 ↔ Nut Thin Nylock:30
- Rigid:217 [WeldJoint]: Nut Thin Nylock:30 ↔ NSpacer .375 OD x .125:25
- [WeldJoint]: Nut Thin Nylock:31 ↔ NSpacer .375 OD x .125:26
- Rigid:219 [WeldJoint]: HS Bearing Flat:5 ↔ Nut Thin Nylock:31
- [WeldJoint]: HS Bearing Flat:6 ↔ Nut Thin Nylock:32
- [WeldJoint]: Nut Thin Nylock:32 ↔ NSpacer .375 OD x .125:27
- [WeldJoint]: Nut Thin Nylock:33 ↔ NSpacer .375 OD x .125:28
- [WeldJoint]: HS Bearing Flat:6 ↔ Nut Thin Nylock:33
- Rigid:224 [WeldJoint]: C-Channel 1x2x1x23:1 ↔ HS Bearing Flat:6
- Rigid:226 [WeldJoint]: C-Channel 1x2x1x23:1 ↔ Nut Thin Nylock:35
- Rigid:228 [WeldJoint]: outer-tower-support-proto:1 ↔ SScrew Star Smooth .875:54
- Rigid:230 [WeldJoint]: outer-tower-support-proto:2 ↔ SScrew Star Smooth .875:56
- Rigid:232 [WeldJoint]: C-Channel 1x2x1x23:2 ↔ Nut Thin Nylock:37
- Rotational:13 [RevoluteJoint] (3.175 mm): C-Channel 1x2x1x23:2 ↔ LS 12T Gear:1
- Rotational:14 [RevoluteJoint] (3.175 mm): C-Channel 1x2x1x23:1 ↔ LS 12T Gear:2
- Rotational:15 [RevoluteJoint]: LS 12T Gear:1 ↔ Nut Thin Nylock:38
- Rotational:16 [RevoluteJoint]: LS 12T Gear:2 ↔ Nut Thin Nylock:39
- Rigid:235 [WeldJoint]: C-Channel 1x2x1x23:1 ↔ NSpacer .375 OD x .125:29
- Rigid:236 [WeldJoint]: C-Channel 1x2x1x23:2 ↔ NSpacer .375 OD x .125:30
- Rigid:237 [WeldJoint]: HSpacer .0625:1 ↔ HSpacer .1250:2
- Rigid:238 [WeldJoint]: HS 12T Gear, No Insert:1 ↔ HSpacer .1250:2
- [WeldJoint]: HSpacer .0625:3 ↔ HSpacer .1250:4
- Rigid:240 [WeldJoint]: HS 12T Gear, No Insert:2 ↔ HSpacer .1250:4
- Rigid:241 [WeldJoint]: outer-tower-support-proto:1 ↔ SScrew Star Smooth 1.500:58
- Rigid:242 [WeldJoint]: outer-tower-support-proto:2 ↔ SScrew Star Smooth 1.500:57
- Rotational:17 [RevoluteJoint] (7.62 mm): HS Bearing Flat:1 ↔ Shaft HS 5.0 in:2
- Rotational:18 [RevoluteJoint] (7.62 mm): HS Bearing Flat:2 ↔ Shaft HS 5.0 in:3
- Rigid:243 [WeldJoint] (-53.2384 mm): HS 12T Gear, No Insert:2 ↔ Shaft HS 5.0 in:3
- Rigid:244 [WeldJoint] (-53.2384 mm): HS 12T Gear, No Insert:1 ↔ Shaft HS 5.0 in:2
- Rigid:245 [WeldJoint] (-10.4648 mm): Shaft HS 5.0 in:3 ↔ 6P 8T Sprocket, No Insert:1
- Rigid:246 [WeldJoint]: HS Bearing Flat:5 ↔ HSpacer .5000:5
- Rigid:247 [WeldJoint]: HSpacer .5000:5 ↔ HSpacer .2500:6
- Rotational:19 [RevoluteJoint]: HSpacer .2500:6 ↔ HSpacer .1250:7
- Rigid:248 [WeldJoint] (-4.1148 mm): Shaft HS 5.0 in:3 ↔ Low Profile HS Shaft Collar:1
- [WeldJoint]: HSpacer .5000:8 ↔ HSpacer .2500:9
- [RevoluteJoint]: HSpacer .2500:9 ↔ HSpacer .1250:10
- Rigid:250 [WeldJoint] (-10.4648 mm): Shaft HS 5.0 in:2 ↔ 6P 8T Sprocket, No Insert:2
- Rigid:251 [WeldJoint]: HS Bearing Flat:6 ↔ HSpacer .5000:8
- Rigid:252 [WeldJoint] (-4.1148 mm): Shaft HS 5.0 in:2 ↔ Low Profile HS Shaft Collar:2
- Rigid:253 [WeldJoint]: HS 12T Gear, No Insert:2 ↔ HSpacer .5000:11
- Rigid:254 [WeldJoint]: HS 12T Gear, No Insert:1 ↔ HSpacer .5000:12
- Rigid:255 [WeldJoint]: HSpacer .5000:11 ↔ Low Profile HS Shaft Collar:3
- Rigid:256 [WeldJoint]: HSpacer .5000:12 ↔ Low Profile HS Shaft Collar:4
- Rigid:257 [WeldJoint]: Low Profile HS Shaft Collar:3 ↔ HSpacer .5000:13
- Rigid:258 [WeldJoint]: HSpacer .5000:13 ↔ HSpacer .1250:14
- Rigid:259 [WeldJoint]: HSpacer .1250:14 ↔ HSpacer .0625:15
- [WeldJoint]: HSpacer .5000:16 ↔ HSpacer .1250:17
- [WeldJoint]: HSpacer .1250:17 ↔ HSpacer .0625:18
- Rigid:262 [WeldJoint]: Low Profile HS Shaft Collar:4 ↔ HSpacer .5000:16
- Rigid:263 [WeldJoint] (12.7 mm): C-Channel 1x2x1x14:1 ↔ L-Channel 1x1x2:3
- Rigid:264 [WeldJoint]: L-Channel 1x1x2:3 ↔ third-stage:1
- Rigid:265 [WeldJoint]: outer-tower-support-proto:2 ↔ first-stage:3
- Rigid:266 [WeldJoint]: outer-tower-support-proto:1 ↔ first-stage:4
## Named parameters: d738_d737 = 0 mm, d739_d737 = 0 mm, d740_d737 = 0 mm, d37_d5 = 0 mm, d38_d6 = 0 mm, d39_d7 = 0 mm, d40_d8 = 0 mm, d1081_d1067_d1065 = 0 mm, d1082_d1068_d1066 = 0 mm, d82_d1081_d1067_d1065 = 0 mm, d83_d1082_d1068_d1066 = 0 mm, d84_d1081_d1067_d1065 = 0 mm, d85_d1082_d1068_d1066 = 0 mm, d86_d1081_d1067_d1065 = 0 mm, d87_d1082_d1068_d1066 = 0 mm, d88_d1081_d1067_d1065 = 0 mm, d89_d1082_d1068_d1066 = 0 mm, d126_d106 = -3.175 mm, d153_d699 = 0 mm, d154_d106 = -3.175 mm, d155_d107 = 3.175 mm, d156_d108 = -137.734545 deg, d157_d114 = 0 mm, d158_d115 = 0 mm, d159_d116 = 0 mm, d160_d117 = 0 mm, d163_d125 = 0 mm, d164_d118 = 0 mm, d165_d119 = 0 mm, d166_d120 = 0 mm, d167_d121 = 0 mm, d168_d122 = 0 mm, d169_d123 = 0 mm, d170_d124 = 0 mm, d177_d140 = 0 mm, d178_d126_d106 = -3.175 mm, d179_d1107 = 0 mm, d180_d1106 = 0 mm, d181_d135 = 0 mm, d182_d136 = 129.863494 deg, d183_d137 = 0 mm, d184_d138 = 0 mm, d185_d139 = 0 mm, d259_d255 = 0 mm, d260_d256 = 0 mm, d261_d258 = 0 mm, d303_d302 = 0 mm, d305_d302 = 0 mm, d306_d303_d302 = 0 mm, d307_d304 = 0 mm, d308_d301 = 0 mm, d336_d334 = 0 mm, d352_d348 = 0 mm, d353_d349 = 0 mm, d354_d350 = 0 deg, d365_d363 = 0 mm, d366_d364 = 0 mm
